# Autodesk Inventor assembly: 20-J2
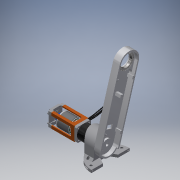
[picture p0: Inventor's stored thumbnail of the model, 180x180]
Saved by Autodesk Inventor 2018 (Build 220112000, 112)
## iProperties
Created: 2020-01-14
Part Number: 20-J2
Document SubType Name: Assembly
Designer: Bunny320
Author: Bunny320
## Documents named in this file (5)
- C:\Users\Bunny320\Desktop\sechs\4-CAD\20-J2.iam
- C:\Users\Bunny320\Desktop\sechs\4-CAD\201-flange-with motor.ipt
- C:\Users\Bunny320\Desktop\sechs\4-CAD\standardParts\61807-2RS1\61807-2RS1.iam
- C:\Users\Bunny320\Desktop\sechs\4-CAD\motor unit.iam
- C:\Users\Bunny320\Desktop\sechs\4-CAD\203-link left.ipt
## Components (5 placed, 4 different names)
1. 201-flange-with motor:1 — Flush:1, Flush:2, Flush:3, Mate:3, Mate:4, Mate:7, Mate:8, Mate:9
2. 61807-2RS1:1 [sub-assembly] — Mate:3, Mate:4, Mate:14
3. motor unit:1 [sub-assembly] — Mate:7, Mate:8, Mate:9, Mate:13
4. 203-link left:1 — Mate:13, Mate:14, Mate:15, Mate:16
5. 61807-2RS1:3 [sub-assembly] — Mate:15, Mate:16
## Relationships (12: Mate 9, Flush 3)
- Flush:1: 201-flange-with motor:1
- Flush:2: 201-flange-with motor:1
- Flush:3: 201-flange-with motor:1
- Mate:3: 201-flange-with motor:1 ↔ 61807-2RS1:1
- Mate:4: 201-flange-with motor:1 ↔ 61807-2RS1:1
- Mate:7: 201-flange-with motor:1 ↔ motor unit:1
- Mate:8: 201-flange-with motor:1 ↔ motor unit:1
- Mate:9: 201-flange-with motor:1 ↔ motor unit:1
- Mate:13: motor unit:1 ↔ 203-link left:1
- Mate:14: 61807-2RS1:1 ↔ 203-link left:1
- Mate:15: 203-link left:1 ↔ 61807-2RS1:3
- Mate:16: 203-link left:1 ↔ 61807-2RS1:3
